# Autodesk Inventor assembly: 組合窗_MIR3
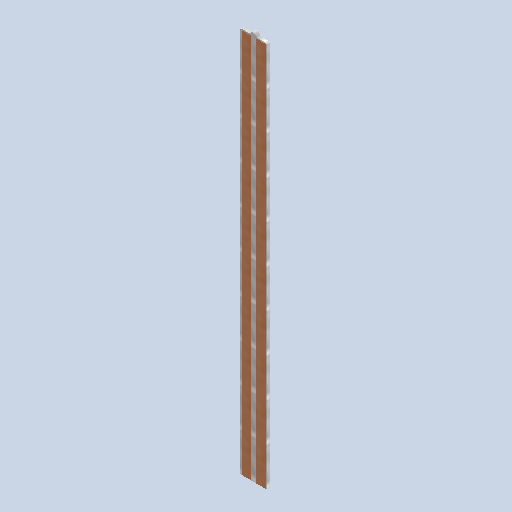
[picture p0: Inventor's stored thumbnail of the model, 512x512]
Saved by Autodesk Inventor 2024.2 (Build 282272000, 272)
## iProperties
Created: 2024-06-01
Part Number: 組合窗_MIR3
Document SubType Name: Assembly
Designer: User
Author: User
## Documents named in this file (5)
- C:\Users\User\OneDrive - 國立中山大學\桌面\創客基礎\final_project\組合窗_MIR3.iam
- C:\Users\User\OneDrive - 國立中山大學\桌面\創客基礎\final_project\窗頂_MIR3.ipt
- C:\Users\User\OneDrive - 國立中山大學\桌面\創客基礎\final_project\窗_MIR3.ipt
- C:\Users\User\OneDrive - 國立中山大學\桌面\創客基礎\final_project\窗間柱_MIR3.ipt
- C:\Users\User\OneDrive - 國立中山大學\桌面\創客基礎\final_project\窗側柱_MIR3.ipt
## Components (51 placed, 4 different names)
1. 窗頂_MIR3:1 — 相切:1, 齊平:9, 貼合:5
2. 窗_MIR3:1 — 齊平:2, 貼合:1, 齊平:1, 齊平:6, 齊平:5, 貼合:3
3. 窗間柱_MIR3:1 — 齊平:2, 貼合:1, 齊平:1, 齊平:4, 齊平:3, 貼合:2, 齊平:9, 貼合:5
4. 窗側柱_MIR3:1 — 齊平:6, 齊平:5, 貼合:3
5. 窗_MIR3:2 — 齊平:4, 齊平:3, 貼合:2, 齊平:8, 齊平:7, 貼合:4
6. 窗側柱_MIR3:2 — 齊平:8, 齊平:7, 貼合:4, 相切:1
7. 窗_MIR3:3
8. 窗間柱_MIR3:2
9. 窗側柱_MIR3:3
10. 窗_MIR3:4
11. 窗側柱_MIR3:4
12. 窗_MIR3:5
13. 窗間柱_MIR3:3
14. 窗側柱_MIR3:5
15. 窗_MIR3:6
16. 窗側柱_MIR3:6
17. 窗_MIR3:7
18. 窗間柱_MIR3:4
19. 窗側柱_MIR3:7
20. 窗_MIR3:8
21. 窗側柱_MIR3:8
22. 窗_MIR3:9
23. 窗間柱_MIR3:5
24. 窗側柱_MIR3:9
25. 窗_MIR3:10
26. 窗側柱_MIR3:10
27. 窗_MIR3:11
28. 窗間柱_MIR3:6
29. 窗側柱_MIR3:11
30. 窗_MIR3:12
31. 窗側柱_MIR3:12
32. 窗_MIR3:13
33. 窗間柱_MIR3:7
34. 窗側柱_MIR3:13
35. 窗_MIR3:14
36. 窗側柱_MIR3:14
37. 窗_MIR3:15
38. 窗間柱_MIR3:8
39. 窗側柱_MIR3:15
40. 窗_MIR3:16
41. 窗側柱_MIR3:16
42. 窗_MIR3:17
43. 窗間柱_MIR3:9
44. 窗側柱_MIR3:17
45. 窗_MIR3:18
46. 窗側柱_MIR3:18
47. 窗_MIR3:19
48. 窗間柱_MIR3:10
49. 窗側柱_MIR3:19
50. 窗_MIR3:20
51. 窗側柱_MIR3:20
## Component patterns: (10 elements, first: 窗_MIR3:1 + 窗間柱_MIR3:1 + 窗側柱_MIR3:1 + 窗_MIR3:2 + 窗側柱_MIR3:2)
## Relationships (15: Flush 9, Mate 5, Tangent 1)
- 齊平:2 [Flush]: 窗_MIR3:1 ↔ 窗間柱_MIR3:1
- 貼合:1 [Mate]: 窗_MIR3:1 ↔ 窗間柱_MIR3:1
- 齊平:1 [Flush]: 窗_MIR3:1 ↔ 窗間柱_MIR3:1
- 齊平:4 [Flush]: 窗間柱_MIR3:1 ↔ 窗_MIR3:2
- 齊平:3 [Flush]: 窗間柱_MIR3:1 ↔ 窗_MIR3:2
- 貼合:2 [Mate]: 窗間柱_MIR3:1 ↔ 窗_MIR3:2
- 齊平:8 [Flush]: 窗_MIR3:2 ↔ 窗側柱_MIR3:2
- 齊平:7 [Flush]: 窗_MIR3:2 ↔ 窗側柱_MIR3:2
- 貼合:4 [Mate]: 窗_MIR3:2 ↔ 窗側柱_MIR3:2
- 齊平:6 [Flush]: 窗_MIR3:1 ↔ 窗側柱_MIR3:1
- 齊平:5 [Flush]: 窗_MIR3:1 ↔ 窗側柱_MIR3:1
- 貼合:3 [Mate]: 窗_MIR3:1 ↔ 窗側柱_MIR3:1
- 相切:1 [Tangent]: 窗頂_MIR3:1 ↔ 窗側柱_MIR3:2
- 齊平:9 [Flush]: 窗頂_MIR3:1 ↔ 窗間柱_MIR3:1
- 貼合:5 [Mate]: 窗頂_MIR3:1 ↔ 窗間柱_MIR3:1
